# Autodesk Inventor assembly: Assembly1
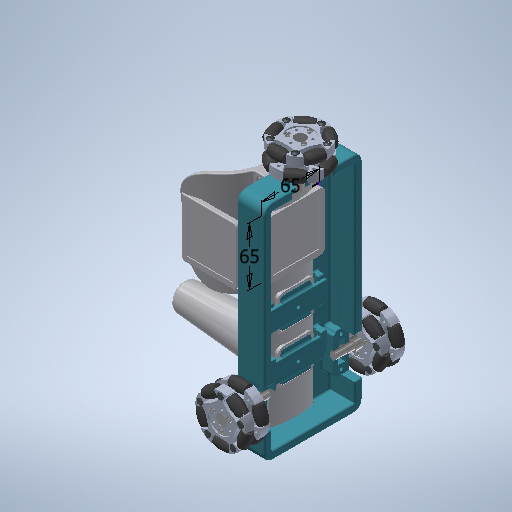
[picture p0: Inventor's stored thumbnail of the model, 512x512]
Saved by Autodesk Inventor 2025 (Build 290162000, 162)
## iProperties
Created: 2024-05-13
Part Number: Assembly1
Document SubType Name: Assembly
Designer: Pintu
Author: Pintu
## Documents named in this file (5)
- D:\CMC\my_inventor\ArmBo_v2\wearable\Assembly1.iam
- D:\CMC\my_inventor\ArmBo_v2\wearable\wearable_old.ipt
- D:\CMC\my_inventor\ArmBo_v2\wearable\new_base_old.ipt
- D:\CMC\my_inventor\ArmBo_v2\support\WheelAsm\WheelAsm.iam
- D:\CMC\my_inventor\ArmBo_v2\new_shaft.ipt
## Components (8 placed, 4 different names)
1. wearable_old:1 — Flush:1, Flush:2, Flush:3, Flush:4
2. new_base_old:1 — Flush:1, Flush:2, Flush:3, Flush:4, Mate:1, Flush:5, Mate:2, Mate:3, Mate:4, Mate:5, Mate:10, Flush:9
3. WheelAsm:1 [sub-assembly] — Mate:8, Flush:7
4. WheelAsm:2 [sub-assembly] — Mate:9, Flush:8
5. WheelAsm:3 [sub-assembly] — Mate:6, Flush:6
6. new_shaft:1 — Mate:1, Flush:5, Mate:9, Flush:8
7. new_shaft:2 — Mate:2, Mate:3, Mate:8, Flush:7, Mate:10, Flush:9
8. new_shaft:3 — Mate:4, Mate:5, Mate:6, Flush:6
## Relationships (18: Flush 9, Mate 9)
- Flush:1: wearable_old:1 ↔ new_base_old:1
- Flush:2: wearable_old:1 ↔ new_base_old:1
- Flush:3: wearable_old:1 ↔ new_base_old:1
- Flush:4: wearable_old:1 ↔ new_base_old:1
- Mate:1: new_base_old:1 ↔ new_shaft:1
- Flush:5: new_base_old:1 ↔ new_shaft:1
- Mate:2: new_base_old:1 ↔ new_shaft:2
- Mate:3: new_base_old:1 ↔ new_shaft:2
- Mate:4: new_base_old:1 ↔ new_shaft:3
- Mate:5: new_base_old:1 ↔ new_shaft:3
- Mate:6: WheelAsm:3 ↔ new_shaft:3
- Flush:6: WheelAsm:3 ↔ new_shaft:3
- Mate:8: WheelAsm:1 ↔ new_shaft:2
- Flush:7: WheelAsm:1 ↔ new_shaft:2
- Mate:9: WheelAsm:2 ↔ new_shaft:1
- Flush:8: WheelAsm:2 ↔ new_shaft:1
- Mate:10: new_base_old:1 ↔ new_shaft:2
- Flush:9: new_base_old:1 ↔ new_shaft:2
